# Autodesk Inventor assembly: ロボハンド
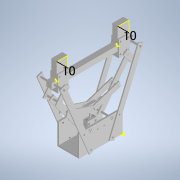
[picture p0: Inventor's stored thumbnail of the model, 180x180]
Saved by Autodesk Inventor 2022 (Build 260153070, 153G)
## iProperties
Created: 2022-09-26
Part Number: ロボハンド
Document SubType Name: Assembly
Designer: hirok
Author: hirok
## Documents named in this file (18)
- C:\Users\hirok\OneDrive\ドキュメント\Inventor\robot_design_2022\ロボハンド.iam
- C:\Users\hirok\OneDrive\ドキュメント\Inventor\robot_design_2022\シリンダー.ipt
- C:\Users\hirok\OneDrive\ドキュメント\Inventor\robot_design_2022\シリンダー棒.ipt
- C:\Users\hirok\OneDrive\ドキュメント\Inventor\robot_design_2022\シリンダーの先に着けるやつ.ipt
- C:\Users\hirok\OneDrive\ドキュメント\Inventor\robot_design_2022\長いほう.ipt
- C:\Users\hirok\OneDrive\ドキュメント\Inventor\robot_design_2022\短い覇王.ipt
- C:\Users\hirok\OneDrive\ドキュメント\Inventor\robot_design_2022\棒.ipt
- C:\Users\hirok\OneDrive\ドキュメント\Inventor\robot_design_2022\棒2.ipt
- C:\Users\hirok\OneDrive\ドキュメント\Inventor\robot_design_2022\指先.ipt
- C:\Users\hirok\OneDrive\ドキュメント\Inventor\robot_design_2022\レール.ipt
- C:\Users\hirok\OneDrive\ドキュメント\Inventor\robot_design_2022\棒３.ipt
- C:\Users\hirok\OneDrive\ドキュメント\Inventor\robot_design_2022\指支え.ipt
- C:\Users\hirok\OneDrive\ドキュメント\Inventor\robot_design_2022\指上.ipt
- C:\Users\hirok\OneDrive\ドキュメント\Inventor\robot_design_2022\指下.ipt
- C:\Users\hirok\OneDrive\ドキュメント\Inventor\robot_design_2021\ベアリング2.ipt
- C:\Users\hirok\OneDrive\ドキュメント\Inventor\robot_design_2022\シリンダーボックス.ipt
- C:\Users\hirok\OneDrive\ドキュメント\Inventor\robot_design_2022\レール接続.ipt
- C:\Users\hirok\OneDrive\ドキュメント\Inventor\robot_design_2022\レール固定.ipt
## Components (59 placed, 17 different names)
1. シリンダー:1 — メイト:1, メイト:2, 挿入:106, 挿入:107
2. シリンダー棒:1 — メイト:1, 挿入:1
3. シリンダーの先に着けるやつ:1 — 挿入:1, 挿入:12, メイト:2, 挿入:55
4. 長いほう:1 — 挿入:11, 挿入:17, 挿入:105
5. 短い覇王:1 — 挿入:9, 挿入:10, 挿入:11, 挿入:12, 挿入:62, 挿入:67
6. 棒:2 — 挿入:9, 挿入:95
7. 棒:5 — 挿入:10, 挿入:94
8. 棒2:1 — 挿入:103
9. 指先:1 — 挿入:17, 挿入:23, 挿入:26, 挿入:58, 挿入:61, 挿入:97
10. 指先:4 — 挿入:24, 挿入:25, 挿入:59, 挿入:60
11. レール:1 — メイト:3, メイト:5, 挿入:116, 挿入:117, 挿入:118
12. 棒３:1 — 挿入:23, 挿入:24
13. 棒３:2 — 挿入:25, 挿入:26
14. 指支え:1 — 挿入:72, 挿入:73, 挿入:74, 挿入:75
15. 指支え:2 — 挿入:70, 挿入:71, 挿入:97
16. 指上:1 — 挿入:74, 挿入:75
17. 指下:1 — 挿入:70, 挿入:71, 挿入:72, 挿入:73, メイト:3
18. 長いほう:2 — 挿入:104
19. 短い覇王:2 — 挿入:55, 挿入:56, 挿入:57
20. 棒:7 — 挿入:93
21. 棒:8 — 挿入:92
22. 指先:5 — 挿入:63, 挿入:64, 挿入:96
23. 指先:6 — 挿入:65, 挿入:66
24. 棒３:3
25. 棒３:4
26. 指支え:5 — 挿入:78, 挿入:79, 挿入:80, 挿入:81
27. 指支え:6 — 挿入:76, 挿入:77, 挿入:96
28. 指上:3 — 挿入:80, 挿入:81, メイト:5
29. 棒2:3 — 挿入:102
30. ベアリング2:1 — 挿入:57
31. ベアリング2:2 — 挿入:56
32. 指下:3 — 挿入:76, 挿入:77, 挿入:78, 挿入:79
33. ベアリング2:3 — 挿入:60
34. ベアリング2:4 — 挿入:63
35. ベアリング2:5 — 挿入:64
36. ベアリング2:6 — 挿入:59
37. ベアリング2:7 — 挿入:65
38. ベアリング2:8 — 挿入:66
39. ベアリング2:9 — 挿入:61
40. ベアリング2:10 — 挿入:58
41. ベアリング2:11 — 挿入:62
42. ベアリング2:12 — 挿入:101
43. ベアリング2:13 — 挿入:67
44. ベアリング2:14 — 挿入:100
45. ベアリング2:15 — 挿入:98
46. ベアリング2:16 — 挿入:99
47. 短い覇王:3 — 挿入:88, 挿入:89, 挿入:94, 挿入:95
48. 短い覇王:4 — 挿入:90, 挿入:91, 挿入:92, 挿入:93
49. ベアリング2:17 — 挿入:90
50. ベアリング2:18 — 挿入:88
51. ベアリング2:19 — 挿入:91
52. ベアリング2:20 — 挿入:89
53. シリンダーボックス:1 — 挿入:98, 挿入:99, 挿入:100, 挿入:101, 挿入:102, 挿入:103, 挿入:104, 挿入:105, 挿入:106, 挿入:107, 挿入:108, 挿入:109, 挿入:110, 挿入:111, 挿入:112, 挿入:113, 挿入:114, 挿入:115
54. レール接続:1 — 挿入:112, 挿入:113, 挿入:118
55. レール接続:2 — 挿入:114, 挿入:115, 挿入:116
56. レール接続:3 — 挿入:108, 挿入:109, 挿入:117, 挿入:120
57. レール接続:4 — 挿入:110, 挿入:111, 挿入:119
58. レール固定:1 — 挿入:120
59. レール固定:2 — 挿入:119
## Relationships (80: Insert 76, Mate 4)
- メイト:1 [Mate]: シリンダー:1 ↔ シリンダー棒:1
- 挿入:1 [Insert]: シリンダー棒:1 ↔ シリンダーの先に着けるやつ:1
- 挿入:9 [Insert]: 短い覇王:1 ↔ 棒:2
- 挿入:10 [Insert]: 短い覇王:1 ↔ 棒:5
- 挿入:11 [Insert] (4 mm): 長いほう:1 ↔ 短い覇王:1
- 挿入:12 [Insert] (2.5 mm): シリンダーの先に着けるやつ:1 ↔ 短い覇王:1
- メイト:2 [Mate] (16 mm): シリンダー:1 ↔ シリンダーの先に着けるやつ:1
- 挿入:17 [Insert] (9.5 mm): 長いほう:1 ↔ 指先:1
- 挿入:23 [Insert]: 指先:1 ↔ 棒３:1
- 挿入:24 [Insert]: 指先:4 ↔ 棒３:1
- 挿入:25 [Insert]: 指先:4 ↔ 棒３:2
- 挿入:26 [Insert]: 指先:1 ↔ 棒３:2
- [Insert]: 短い覇王:2 ↔ 棒:7
- [Insert]: 短い覇王:2 ↔ 棒:8
- [Insert] (4 mm): 長いほう:2 ↔ 短い覇王:2
- [Insert] (9.5 mm): 長いほう:2 ↔ 指先:5
- [Insert]: 指先:5 ↔ 棒３:3
- [Insert]: 指先:6 ↔ 棒３:3
- [Insert]: 指先:6 ↔ 棒３:4
- [Insert]: 指先:5 ↔ 棒３:4
- 挿入:55 [Insert] (2.5 mm): シリンダーの先に着けるやつ:1 ↔ 短い覇王:2
- 挿入:56 [Insert]: 短い覇王:2 ↔ ベアリング2:2
- 挿入:57 [Insert]: 短い覇王:2 ↔ ベアリング2:1
- 挿入:58 [Insert]: 指先:1 ↔ ベアリング2:10
- 挿入:59 [Insert]: 指先:4 ↔ ベアリング2:6
- 挿入:60 [Insert]: 指先:4 ↔ ベアリング2:3
- 挿入:61 [Insert]: 指先:1 ↔ ベアリング2:9
- 挿入:62 [Insert]: 短い覇王:1 ↔ ベアリング2:11
- 挿入:63 [Insert]: 指先:5 ↔ ベアリング2:4
- 挿入:64 [Insert]: 指先:5 ↔ ベアリング2:5
- 挿入:65 [Insert]: 指先:6 ↔ ベアリング2:7
- 挿入:66 [Insert]: 指先:6 ↔ ベアリング2:8
- 挿入:67 [Insert]: 短い覇王:1 ↔ ベアリング2:13
- 挿入:70 [Insert]: 指支え:2 ↔ 指下:1
- 挿入:71 [Insert]: 指支え:2 ↔ 指下:1
- 挿入:72 [Insert]: 指支え:1 ↔ 指下:1
- 挿入:73 [Insert]: 指支え:1 ↔ 指下:1
- 挿入:74 [Insert]: 指支え:1 ↔ 指上:1
- 挿入:75 [Insert]: 指支え:1 ↔ 指上:1
- 挿入:76 [Insert]: 指支え:6 ↔ 指下:3
- 挿入:77 [Insert]: 指支え:6 ↔ 指下:3
- 挿入:78 [Insert]: 指支え:5 ↔ 指下:3
- 挿入:79 [Insert]: 指支え:5 ↔ 指下:3
- 挿入:80 [Insert]: 指支え:5 ↔ 指上:3
- 挿入:81 [Insert]: 指支え:5 ↔ 指上:3
- メイト:3 [Mate]: レール:1 ↔ 指下:1
- メイト:5 [Mate]: レール:1 ↔ 指上:3
- 挿入:88 [Insert]: 短い覇王:3 ↔ ベアリング2:18
- 挿入:89 [Insert]: 短い覇王:3 ↔ ベアリング2:20
- 挿入:90 [Insert]: 短い覇王:4 ↔ ベアリング2:17
- 挿入:91 [Insert]: 短い覇王:4 ↔ ベアリング2:19
- 挿入:92 [Insert]: 棒:8 ↔ 短い覇王:4
- 挿入:93 [Insert]: 棒:7 ↔ 短い覇王:4
- 挿入:94 [Insert]: 棒:5 ↔ 短い覇王:3
- 挿入:95 [Insert]: 棒:2 ↔ 短い覇王:3
- 挿入:96 [Insert] (3.5 mm): 指先:5 ↔ 指支え:6
- 挿入:97 [Insert] (3.5 mm): 指先:1 ↔ 指支え:2
- 挿入:98 [Insert]: ベアリング2:15 ↔ シリンダーボックス:1
- 挿入:99 [Insert]: ベアリング2:16 ↔ シリンダーボックス:1
- 挿入:100 [Insert]: ベアリング2:14 ↔ シリンダーボックス:1
- 挿入:101 [Insert]: ベアリング2:12 ↔ シリンダーボックス:1
- 挿入:102 [Insert]: 棒2:3 ↔ シリンダーボックス:1
- 挿入:103 [Insert]: 棒2:1 ↔ シリンダーボックス:1
- 挿入:104 [Insert] (16 mm): 長いほう:2 ↔ シリンダーボックス:1
- 挿入:105 [Insert] (16 mm): 長いほう:1 ↔ シリンダーボックス:1
- 挿入:106 [Insert] (13 mm): シリンダー:1 ↔ シリンダーボックス:1
- 挿入:107 [Insert] (13 mm): シリンダー:1 ↔ シリンダーボックス:1
- 挿入:108 [Insert]: シリンダーボックス:1 ↔ レール接続:3
- 挿入:109 [Insert]: シリンダーボックス:1 ↔ レール接続:3
- 挿入:110 [Insert]: シリンダーボックス:1 ↔ レール接続:4
- 挿入:111 [Insert]: シリンダーボックス:1 ↔ レール接続:4
- 挿入:112 [Insert]: シリンダーボックス:1 ↔ レール接続:1
- 挿入:113 [Insert]: シリンダーボックス:1 ↔ レール接続:1
- 挿入:114 [Insert]: シリンダーボックス:1 ↔ レール接続:2
- 挿入:115 [Insert]: シリンダーボックス:1 ↔ レール接続:2
- 挿入:116 [Insert] (15 mm): レール:1 ↔ レール接続:2
- 挿入:117 [Insert] (15 mm): レール:1 ↔ レール接続:3
- 挿入:118 [Insert] (15 mm): レール:1 ↔ レール接続:1
- 挿入:119 [Insert] (-3 mm): レール接続:4 ↔ レール固定:2
- 挿入:120 [Insert] (-3 mm): レール接続:3 ↔ レール固定:1
## Named parameters: d47_d9 = 0 mm, d48_d10 = 0 mm, d49_d11 = 4 mm, d53_d21 = 9.5 mm, d54_d32 = 0 mm, d59_d27 = 0 mm, d60_d29 = 0 mm, d61_d31 = 0 mm
